# Autodesk Inventor assembly: AX-03_Assembly
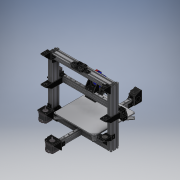
[picture p0: Inventor's stored thumbnail of the model, 180x180]
Saved by Autodesk Inventor 2017.3 (Build 213256000, 256)
## iProperties
Created: 2018-09-09
Part Number: AX-03_Assembly
Document SubType Name: Assembly
Designer: Ax
Author: Ax
## Documents named in this file (41)
- C:\Users\Ax\Documents\Inventor\AX-03\AX-03_Assembly.iam
- C:\Users\Ax\Documents\Inventor\AX-03\Endstop2.iam
- C:\Users\Ax\Documents\Inventor\AX-03\GT2_20T.ipt
- C:\Users\Ax\Documents\Inventor\AX-03\NFS5-2020-340.ipt
- C:\Users\Ax\Documents\Inventor\AX-03\NFS5-2020-400.ipt
- C:\Users\Ax\Documents\Inventor\AX-03\NFS5-2040-140.ipt
- C:\Users\Ax\Documents\Inventor\AX-03\NFS5-2040-300.ipt
- C:\Users\Ax\Documents\Inventor\AX-03\SEBZ13-295.iam
- C:\Users\Ax\Documents\Inventor\AX-03\SSEB10-295.iam
- C:\Users\Ax\Documents\Inventor\AX-03\SSEBZ13-395.iam
- C:\Users\Ax\Documents\Inventor\AX-03\NFS5-2040-300_CPY.ipt
- C:\Users\Ax\Documents\Inventor\AX-03\NFS5-2040-140_CPY.ipt
- C:\Users\Ax\Documents\Inventor\AX-03\SSEB10-295_CPY.iam
- C:\Users\Ax\Documents\Inventor\AX-03\Main_Frame_Bracket.ipt
- C:\Users\Ax\Documents\Inventor\AX-03\X_Z_Axis_Left.ipt
- C:\Users\Ax\Documents\Inventor\AX-03\X_Z_Axis_Right_-_add_meat_to_Endstop_contact.ipt
- C:\Users\Ax\Documents\Inventor\AX-03\Y_Motor_Holder001.ipt
- C:\Users\Ax\Documents\Inventor\AX-03\Bed_Carrier001.ipt
- C:\Users\Ax\Documents\Inventor\AX-03\Z_Motor_Holder001.ipt
- C:\Users\Ax\Documents\Inventor\AX-03\Z_Belt_Tensioner.iam
- C:\Users\Ax\Documents\Inventor\AX-03\Y_Belt_Tensioner_End.ipt
- C:\Users\Ax\Documents\Inventor\AX-03\Y_Belt_Clip001.ipt
- C:\Users\Ax\Documents\Inventor\AX-03\Z_Leadscrew_Bearing_Mount.ipt
- C:\Users\Ax\Documents\Inventor\Content Center Files\R2017\en-US\JIS B 1521 SKF (E)\JIS B 1521 SKF (E) - SKF 608-2Z.ipt
- C:\Users\Ax\Documents\Git\AX-03-Railgun\FreeCAD\STEP\17HS08-1004S.ipt
- C:\Users\Ax\Documents\Inventor\AX-03\PM Wantai 609  Nema 17.ipt
- C:\Users\Ax\Documents\Inventor\AX-03\PM Wantai 609  Nema 17_CPY.ipt
- C:\Users\Ax\Documents\Inventor\AX-03\Extruder_Mount.ipt
- C:\Users\Ax\Documents\Inventor\AX-03\X_Belt_Clip001.ipt
- C:\Users\Ax\Documents\Inventor\AX-03\Drakon.ipt
- C:\Users\Ax\Documents\Inventor\AX-03\E3Dv6.ipt
- C:\Users\Ax\Documents\Inventor\AX-03\30mm_clip_with_venturi_v3_50.ipt
- C:\Users\Ax\Documents\Inventor\AX-03\5015_left-handed_layer_cooling_adapter_-_for_prusa_cooler_v1_21.ipt
- C:\Users\Ax\Documents\Inventor\AX-03\prusa_nozzle_fan_converted_2_v3_4.ipt
- C:\Users\Ax\Documents\Inventor\AX-03\Radial-Cooling-Fan-5015-DC12V.ipt
- C:\Users\Ax\Documents\Inventor\AX-03\30mm Fan.ipt
- C:\Users\Ax\Documents\Inventor\AX-03\Y_Idler.ipt
- C:\Users\Ax\Documents\Inventor\AX-03\X_Idler.ipt
- C:\Users\Ax\Documents\Inventor\AX-03\Leadscrew_Top_Support_Left.ipt
- C:\Users\Ax\Documents\Inventor\AX-03\Leadscrew_Top_Support_Right.ipt
- C:\Users\Ax\Documents\Inventor\AX-03\Bed_Plate.ipt
## Components (46 placed, 40 different names)
1. Endstop2:1 [sub-assembly]
2. GT2_20T:1 — Mate:100, Mate:101
3. Main_Frame_Bracket:1 — Flush:23, Mate:19, Mate:20
4. Main_Frame_Bracket:2 — Flush:32, Mate:27, Flush:33, Mate:32
5. Main_Frame_Bracket:3 — Flush:30, Mate:25, Mate:31
6. Main_Frame_Bracket:4 — Flush:31, Mate:26, Mate:33
7. X_Z_Axis_Left:1 — Mate:37, Mate:38, Mate:39, Mate:41, Mate:42, Mate:43, Mate:44, Mate:119, Mate:120
8. X_Z_Axis_Right:1 — Mate:34, Mate:35, Mate:36, Mate:40, Mate:72, Mate:73, Mate:74
9. Y_Motor_Holder001:1 — Flush:35, Mate:46, Mate:47, Mate:69, Mate:70, Mate:71
10. Bed_Carrier001:1 — Mate:48, Mate:49, Mate:50, Mate:58, Mate:59, Mate:60, Mate:61, Mate:62, Mate:63, Mate:123, Mate:124, Mate:125
11. Z_Motor_Holder001:1 — Flush:36, Mate:54, Flush:37, Mate:75, Mate:76, Mate:77
12. Z_Belt_Tensioner:1 [sub-assembly] — Flush:38, Mate:55
13. Y_Belt_Tensioner_End:1 — Mate:56, Flush:39, Mate:57, Mate:117, Mate:118
14. Y_Belt_Clip001:1 — Mate:61, Mate:62, Mate:63
15. Y_Belt_Clip001:2 — Mate:58, Mate:59, Mate:60
16. Z_Leadscrew_Bearing_Mount:1 — Mate:66, Mate:67, Mate:68, Flush:44
17. JIS B 1521 SKF- with two Z shields SKF 608-2Z:1 — Mate:68, Flush:44
18. 17HS08-1004S:1 — Mate:87, Mate:88, Mate:89, Mate:90
19. PM Wantai 609  Nema 17:1 — Mate:69, Mate:70, Mate:71
20. PM Wantai 609  Nema 17:2 — Mate:72, Mate:73, Mate:74, Mate:100, Mate:101
21. PM Wantai 609  Nema 17_CPY:1 — Mate:75, Mate:76, Mate:77
22. Extruder_Mount:1 — Mate:81, Mate:82, Mate:83, Mate:87, Mate:88, Mate:89, Mate:90, Mate:91, Mate:92, Mate:93, Mate:94, Mate:97, Mate:98, Mate:99
23. X_Belt_Clip001:1 — Mate:81, Mate:82, Mate:83
24. Drakon:1 — Mate:91, Mate:92, Mate:93, Mate:94, Mate:106, Mate:107
25. E3Dv6:1 — Mate:102, Flush:45, Mate:106, Mate:107
26. 30mm_clip_with_venturi_v3_50:1 — Mate:102, Flush:45, Mate:103, Mate:104, Mate:105, Mate:114, Mate:115, Mate:116
27. 5015_left-handed_layer_cooling_adapter_-_for_prusa_cooler_v1_21:1 — Mate:103, Mate:104, Mate:105, Mate:108, Mate:109, Mate:110, Mate:111, Mate:112, Mate:113
28. prusa_nozzle_fan_converted_2_v3_4:1 — Mate:108, Mate:109, Mate:110
29. Radial-Cooling-Fan-5015-DC12V:1 — Mate:111, Mate:112, Mate:113
30. 30mm Fan:1 — Mate:114, Mate:115, Mate:116
31. Y_Idler:1 — Mate:117, Mate:118
32. X_Idler:1 — Mate:119, Mate:120
33. Leadscrew_Top_Support_Left:1 — Mate:121, Flush:46, Flush:47
34. Leadscrew_Top_Support_Right:1 — Mate:122, Flush:48, Flush:49
35. Bed_Plate:1 — Mate:123, Mate:124, Mate:125
36. SSEB10-295_CPY:1 [sub-assembly] — Flush:21, Mate:17, Flush:22, Mate:18, Mate:34, Mate:35
37. SEBZ13-295:1 [sub-assembly] — Mate:43, Flush:34, Mate:45, Mate:97, Mate:98, Mate:99
38. SSEB10-295:1 [sub-assembly] — Mate:12, Mate:13, Flush:9, Mate:37, Mate:38
39. SSEBZ13-395:1 [sub-assembly] — Mate:10, Flush:8, Mate:11, Mate:48, Mate:49, Mate:50
40. NFS5-2040-300_CPY:2 — Flush:14, Flush:15, Mate:15, Mate:16, Flush:16, Flush:19, Flush:21, Mate:17, Flush:22, Mate:18, Flush:33, Mate:36, Mate:54, Flush:37, Mate:122, Flush:48
41. NFS5-2040-140_CPY:1 — Flush:10, Flush:11, Flush:12, Flush:13, Mate:14, Flush:14, Flush:15, Mate:15, Flush:23, Mate:19, Mate:20, Flush:36
42. NFS5-2020-340:1 — Mate:40, Mate:41, Mate:42, Flush:34, Mate:44, Mate:45
43. NFS5-2020-400:1 — Mate:3, Mate:4, Flush:2, Mate:10, Flush:8, Mate:11, Flush:12, Mate:14, Flush:35, Mate:46, Mate:47, Mate:56, Flush:39, Mate:57
44. NFS5-2040-140:1 — Flush:1, Mate:3, Mate:4, Flush:2, Flush:10, Flush:11, Flush:13, Flush:27, Flush:29, Mate:23, Flush:30, Mate:25, Mate:31
45. NFS5-2040-300:1 — Flush:1, Mate:12, Mate:13, Flush:9, Flush:17, Flush:18, Flush:20, Flush:26, Flush:27, Flush:28, Flush:29, Mate:22, Mate:23, Flush:31, Mate:39, Mate:66, Mate:67, Mate:121, Flush:46
46. NFS5-2040-300_CPY:1 — Mate:16, Flush:16, Flush:17, Flush:18, Flush:19, Flush:20, Flush:26, Flush:28, Mate:22, Mate:26, Flush:32, Mate:27, Mate:32, Mate:33, Flush:38, Mate:55, Flush:47, Flush:49
## Relationships (138: Mate 100, Flush 38)
- Flush:1: NFS5-2040-140:1 ↔ NFS5-2040-300:1
- Mate:3: NFS5-2020-400:1 ↔ NFS5-2040-140:1
- Mate:4 (240 mm): NFS5-2020-400:1 ↔ NFS5-2040-140:1
- Flush:2: NFS5-2020-400:1 ↔ NFS5-2040-140:1
- Mate:10 (2.5 mm): SSEBZ13-395:1 ↔ NFS5-2020-400:1
- Flush:8 (4 mm): SSEBZ13-395:1 ↔ NFS5-2020-400:1
- Mate:11 (2.5 mm): SSEBZ13-395:1 ↔ NFS5-2020-400:1
- Mate:12: SSEB10-295:1 ↔ NFS5-2040-300:1
- Mate:13 (5 mm): SSEB10-295:1 ↔ NFS5-2040-300:1
- Flush:9 (5 mm): SSEB10-295:1 ↔ NFS5-2040-300:1
- Flush:10: NFS5-2040-140_CPY:1 ↔ NFS5-2040-140:1
- Flush:11: NFS5-2040-140_CPY:1 ↔ NFS5-2040-140:1
- Flush:12: NFS5-2040-140_CPY:1 ↔ NFS5-2020-400:1
- Flush:13: NFS5-2040-140_CPY:1 ↔ NFS5-2040-140:1
- Mate:14 (1 mm): NFS5-2040-140_CPY:1 ↔ NFS5-2020-400:1
- Flush:14: NFS5-2040-300_CPY:2 ↔ NFS5-2040-140_CPY:1
- Flush:15: NFS5-2040-300_CPY:2 ↔ NFS5-2040-140_CPY:1
- Mate:15: NFS5-2040-300_CPY:2 ↔ NFS5-2040-140_CPY:1
- Mate:16: NFS5-2040-300_CPY:2 ↔ NFS5-2040-300_CPY:1
- Flush:16: NFS5-2040-300_CPY:2 ↔ NFS5-2040-300_CPY:1
- Flush:17: NFS5-2040-300:1 ↔ NFS5-2040-300_CPY:1
- Flush:18: NFS5-2040-300:1 ↔ NFS5-2040-300_CPY:1
- Flush:19: NFS5-2040-300_CPY:2 ↔ NFS5-2040-300_CPY:1
- Flush:20: NFS5-2040-300:1 ↔ NFS5-2040-300_CPY:1
- Flush:21: SSEB10-295_CPY:1 ↔ NFS5-2040-300_CPY:2
- Mate:17: SSEB10-295_CPY:1 ↔ NFS5-2040-300_CPY:2
- Flush:22 (5 mm): SSEB10-295_CPY:1 ↔ NFS5-2040-300_CPY:2
- Mate:18 (5 mm): SSEB10-295_CPY:1 ↔ NFS5-2040-300_CPY:2
- Flush:23: Main_Frame_Bracket:1 ↔ NFS5-2040-140_CPY:1
- Mate:19: Main_Frame_Bracket:1 ↔ NFS5-2040-140_CPY:1
- Mate:20: Main_Frame_Bracket:1 ↔ NFS5-2040-140_CPY:1
- Flush:26: NFS5-2040-300:1 ↔ NFS5-2040-300_CPY:1
- Flush:27: NFS5-2040-140:1 ↔ NFS5-2040-300:1
- Flush:28: NFS5-2040-300:1 ↔ NFS5-2040-300_CPY:1
- Flush:29: NFS5-2040-140:1 ↔ NFS5-2040-300:1
- Mate:22: NFS5-2040-300:1 ↔ NFS5-2040-300_CPY:1
- Mate:23: NFS5-2040-140:1 ↔ NFS5-2040-300:1
- Flush:30: Main_Frame_Bracket:3 ↔ NFS5-2040-140:1
- Mate:25: Main_Frame_Bracket:3 ↔ NFS5-2040-140:1
- Flush:31: Main_Frame_Bracket:4 ↔ NFS5-2040-300:1
- Mate:26: Main_Frame_Bracket:4 ↔ NFS5-2040-300_CPY:1
- Flush:32: Main_Frame_Bracket:2 ↔ NFS5-2040-300_CPY:1
- Mate:27: Main_Frame_Bracket:2 ↔ NFS5-2040-300_CPY:1
- Flush:33: Main_Frame_Bracket:2 ↔ NFS5-2040-300_CPY:2
- Mate:31: Main_Frame_Bracket:3 ↔ NFS5-2040-140:1
- Mate:32: Main_Frame_Bracket:2 ↔ NFS5-2040-300_CPY:1
- Mate:33: Main_Frame_Bracket:4 ↔ NFS5-2040-300_CPY:1
- Mate:34: X_Z_Axis_Right:1 ↔ SSEB10-295_CPY:1
- Mate:35: X_Z_Axis_Right:1 ↔ SSEB10-295_CPY:1
- Mate:36 (0.5 mm): X_Z_Axis_Right:1 ↔ NFS5-2040-300_CPY:2
- Mate:37: X_Z_Axis_Left:1 ↔ SSEB10-295:1
- Mate:38: X_Z_Axis_Left:1 ↔ SSEB10-295:1
- Mate:39 (0.5 mm): X_Z_Axis_Left:1 ↔ NFS5-2040-300:1
- Mate:40: X_Z_Axis_Right:1 ↔ NFS5-2020-340:1
- Mate:41: X_Z_Axis_Left:1 ↔ NFS5-2020-340:1
- Mate:42: X_Z_Axis_Left:1 ↔ NFS5-2020-340:1
- Mate:43 (2.5 mm): X_Z_Axis_Left:1 ↔ SEBZ13-295:1
- Flush:34 (4 mm): SEBZ13-295:1 ↔ NFS5-2020-340:1
- Mate:44: X_Z_Axis_Left:1 ↔ NFS5-2020-340:1
- Mate:45: SEBZ13-295:1 ↔ NFS5-2020-340:1
- Flush:35: Y_Motor_Holder001:1 ↔ NFS5-2020-400:1
- Mate:46: Y_Motor_Holder001:1 ↔ NFS5-2020-400:1
- Mate:47: Y_Motor_Holder001:1 ↔ NFS5-2020-400:1
- Mate:48: Bed_Carrier001:1 ↔ SSEBZ13-395:1
- Mate:49: Bed_Carrier001:1 ↔ SSEBZ13-395:1
- Mate:50: Bed_Carrier001:1 ↔ SSEBZ13-395:1
- Flush:36: Z_Motor_Holder001:1 ↔ NFS5-2040-140_CPY:1
- Mate:54: Z_Motor_Holder001:1 ↔ NFS5-2040-300_CPY:2
- Flush:37: Z_Motor_Holder001:1 ↔ NFS5-2040-300_CPY:2
- Flush:38: Z_Belt_Tensioner:1 ↔ NFS5-2040-300_CPY:1
- Mate:55: Z_Belt_Tensioner:1 ↔ NFS5-2040-300_CPY:1
- Mate:56: Y_Belt_Tensioner_End:1 ↔ NFS5-2020-400:1
- Flush:39: Y_Belt_Tensioner_End:1 ↔ NFS5-2020-400:1
- Mate:57: Y_Belt_Tensioner_End:1 ↔ NFS5-2020-400:1
- Mate:58: Bed_Carrier001:1 ↔ Y_Belt_Clip001:2
- Mate:59: Bed_Carrier001:1 ↔ Y_Belt_Clip001:2
- Mate:60: Bed_Carrier001:1 ↔ Y_Belt_Clip001:2
- Mate:61: Bed_Carrier001:1 ↔ Y_Belt_Clip001:1
- Mate:62: Bed_Carrier001:1 ↔ Y_Belt_Clip001:1
- Mate:63: Bed_Carrier001:1 ↔ Y_Belt_Clip001:1
- Mate:66: Z_Leadscrew_Bearing_Mount:1 ↔ NFS5-2040-300:1
- Mate:67: Z_Leadscrew_Bearing_Mount:1 ↔ NFS5-2040-300:1
- Mate:68: Z_Leadscrew_Bearing_Mount:1 ↔ JIS B 1521 SKF- with two Z shields SKF 608-2Z:1
- Flush:44: Z_Leadscrew_Bearing_Mount:1 ↔ JIS B 1521 SKF- with two Z shields SKF 608-2Z:1
- Mate:69: Y_Motor_Holder001:1 ↔ PM Wantai 609  Nema 17:1
- Mate:70: Y_Motor_Holder001:1 ↔ PM Wantai 609  Nema 17:1
- Mate:71: Y_Motor_Holder001:1 ↔ PM Wantai 609  Nema 17:1
- Mate:72: X_Z_Axis_Right:1 ↔ PM Wantai 609  Nema 17:2
- Mate:73: X_Z_Axis_Right:1 ↔ PM Wantai 609  Nema 17:2
- Mate:74: X_Z_Axis_Right:1 ↔ PM Wantai 609  Nema 17:2
- Mate:75: Z_Motor_Holder001:1 ↔ PM Wantai 609  Nema 17_CPY:1
- Mate:76: Z_Motor_Holder001:1 ↔ PM Wantai 609  Nema 17_CPY:1
- Mate:77: Z_Motor_Holder001:1 ↔ PM Wantai 609  Nema 17_CPY:1
- Mate:81: Extruder_Mount:1 ↔ X_Belt_Clip001:1
- Mate:82: Extruder_Mount:1 ↔ X_Belt_Clip001:1
- Mate:83: Extruder_Mount:1 ↔ X_Belt_Clip001:1
- Mate:87: 17HS08-1004S:1 ↔ Extruder_Mount:1
- Mate:88: 17HS08-1004S:1 ↔ Extruder_Mount:1
- Mate:89: 17HS08-1004S:1 ↔ Extruder_Mount:1
- Mate:90: 17HS08-1004S:1 ↔ Extruder_Mount:1
- Mate:91: Extruder_Mount:1 ↔ Drakon:1
- Mate:92: Extruder_Mount:1 ↔ Drakon:1
- Mate:93: Extruder_Mount:1 ↔ Drakon:1
- Mate:94: Extruder_Mount:1 ↔ Drakon:1
- Mate:97: Extruder_Mount:1 ↔ SEBZ13-295:1
- Mate:98: Extruder_Mount:1 ↔ SEBZ13-295:1
- Mate:99: Extruder_Mount:1 ↔ SEBZ13-295:1
- Mate:100: GT2_20T:1 ↔ PM Wantai 609  Nema 17:2
- Mate:101: GT2_20T:1 ↔ PM Wantai 609  Nema 17:2
- Mate:102: E3Dv6:1 ↔ 30mm_clip_with_venturi_v3_50:1
- Flush:45: E3Dv6:1 ↔ 30mm_clip_with_venturi_v3_50:1
- Mate:103: 30mm_clip_with_venturi_v3_50:1 ↔ 5015_left-handed_layer_cooling_adapter_-_for_prusa_cooler_v1_21:1
- Mate:104: 30mm_clip_with_venturi_v3_50:1 ↔ 5015_left-handed_layer_cooling_adapter_-_for_prusa_cooler_v1_21:1
- Mate:105: 30mm_clip_with_venturi_v3_50:1 ↔ 5015_left-handed_layer_cooling_adapter_-_for_prusa_cooler_v1_21:1
- Mate:106: Drakon:1 ↔ E3Dv6:1
- Mate:107: Drakon:1 ↔ E3Dv6:1
- Mate:108: 5015_left-handed_layer_cooling_adapter_-_for_prusa_cooler_v1_21:1 ↔ prusa_nozzle_fan_converted_2_v3_4:1
- Mate:109: 5015_left-handed_layer_cooling_adapter_-_for_prusa_cooler_v1_21:1 ↔ prusa_nozzle_fan_converted_2_v3_4:1
- Mate:110: 5015_left-handed_layer_cooling_adapter_-_for_prusa_cooler_v1_21:1 ↔ prusa_nozzle_fan_converted_2_v3_4:1
- Mate:111: 5015_left-handed_layer_cooling_adapter_-_for_prusa_cooler_v1_21:1 ↔ Radial-Cooling-Fan-5015-DC12V:1
- Mate:112: 5015_left-handed_layer_cooling_adapter_-_for_prusa_cooler_v1_21:1 ↔ Radial-Cooling-Fan-5015-DC12V:1
- Mate:113: 5015_left-handed_layer_cooling_adapter_-_for_prusa_cooler_v1_21:1 ↔ Radial-Cooling-Fan-5015-DC12V:1
- Mate:114: 30mm_clip_with_venturi_v3_50:1 ↔ 30mm Fan:1
- Mate:115: 30mm_clip_with_venturi_v3_50:1 ↔ 30mm Fan:1
- Mate:116: 30mm_clip_with_venturi_v3_50:1 ↔ 30mm Fan:1
- Mate:117: Y_Belt_Tensioner_End:1 ↔ Y_Idler:1
- Mate:118: Y_Belt_Tensioner_End:1 ↔ Y_Idler:1
- Mate:119: X_Z_Axis_Left:1 ↔ X_Idler:1
- Mate:120: X_Z_Axis_Left:1 ↔ X_Idler:1
- Mate:121: Leadscrew_Top_Support_Left:1 ↔ NFS5-2040-300:1
- Flush:46: Leadscrew_Top_Support_Left:1 ↔ NFS5-2040-300:1
- Flush:47: Leadscrew_Top_Support_Left:1 ↔ NFS5-2040-300_CPY:1
- Mate:122: Leadscrew_Top_Support_Right:1 ↔ NFS5-2040-300_CPY:2
- Flush:48: Leadscrew_Top_Support_Right:1 ↔ NFS5-2040-300_CPY:2
- Flush:49: Leadscrew_Top_Support_Right:1 ↔ NFS5-2040-300_CPY:1
- Mate:123 (20 mm): Bed_Carrier001:1 ↔ Bed_Plate:1
- Mate:124: Bed_Carrier001:1 ↔ Bed_Plate:1
- Mate:125: Bed_Carrier001:1 ↔ Bed_Plate:1
